# Autodesk Inventor assembly: arpans version robot
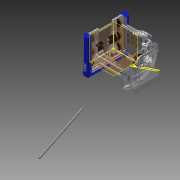
[picture p0: Inventor's stored thumbnail of the model, 180x180]
Saved by Autodesk Inventor 2013 (Build 170138000, 138)
## iProperties
Created: 2013-01-06
Part Number: arpans version robot
Document SubType Name: Assembly
Designer: Moses
Mass: 53939.9 g
Surface Area: 135947 cm^2
Volume: 43150 cm^3
Density: 1.25005 g/cm^3
Author: Moses
## Documents named in this file (39)
- C:\Users\Arpan\Documents\GitHub\frc2013CAD\arpans version robot.iam
- C:\Users\Arpan\Documents\GitHub\frc2013CAD\Drivetrain\Bearings\fr8zz-hex.ipt
- C:\Users\Arpan\Documents\GitHub\frc2013CAD\Drivetrain\Drive Wheel Assembly V2.iam
- C:\Users\Arpan\Documents\GitHub\frc2013CAD\Drivetrain\Standard Wheel Assembly V2.iam
- C:\Users\Arpan\Documents\GitHub\frc2013CAD\Drivetrain\Toughbox-mini\Toughbox-mini-hex-long.iam
- C:\Users\Arpan\Documents\GitHub\frc2013CAD\Drivetrain\6157K140 Shaft Collar\6157K140.ipt
- C:\Users\Arpan\Documents\GitHub\frc2013CAD\Drivetrain\Shaft Spacer Part1.ipt
- C:\Users\Arpan\Documents\GitHub\frc2013CAD\Drivetrain\Shaft Spacer Part2.ipt
- C:\Users\Arpan\Documents\GitHub\frc2013CAD\Drivetrain\Shaft Spacer Part3.ipt
- C:\Users\Arpan\Documents\GitHub\frc2013CAD\Drivetrain\Shaft Spacer Part4.ipt
- C:\Users\Arpan\Documents\GitHub\frc2013CAD\Drivetrain\Shaft Spacer Part5.ipt
- C:\Users\Arpan\Documents\GitHub\frc2013CAD\Drivetrain\Shaft Spacer Part6.ipt
- C:\Users\Arpan\Documents\GitHub\frc2013CAD\Drivetrain\6061K130 Shaft\6061K130.ipt
- C:\Users\Arpan\Documents\GitHub\frc2013CAD\Electrical\CS_compactRIO_cRIO-FRC-II.ipt
- C:\Users\Arpan\Documents\GitHub\frc2013CAD\Electrical\CS_WirelessBridge_DAP1522.ipt
- C:\Users\Arpan\Documents\GitHub\frc2013CAD\Drivetrain\Pneumatic_Compressor_VIAIR_00090\Pneumatic_Compressor_VIAIR_00090.iam
- C:\Users\Arpan\Documents\GitHub\frc2013CAD\Drivetrain\Mounting Bracket V1.500 - (toughbox-mini - sheet metal).ipt
- C:\Users\Arpan\Documents\GitHub\frc2013CAD\Drivetrain\Mounting Bracket V1.500 - (toughbox-mini - sheet metal - underside).ipt
- C:\Users\Arpan\Documents\GitHub\frc2013CAD\Drivetrain\Bearing Block V1.500 Drivetrain.ipt
- C:\Users\Arpan\Documents\GitHub\frc2013CAD\Drivetrain\Shaft Mount V1.500 Drivetrain.ipt
- C:\Users\Arpan\Documents\GitHub\frc2013CAD\Launcher\Shooter\Shooter Assembly v2.iam
- C:\Users\Arpan\Documents\GitHub\frc2013CAD\Chassis\Chassis Assembly 26x28 Version\Chassis Assembly 26x28 Version.iam
- C:\Users\Arpan\Documents\GitHub\frc2013CAD\Chassis\Bumpers\Bumper Assembly1 (26x28 robot).iam
- C:\Users\Arpan\Documents\GitHub\frc2013CAD\Electrical\Mounting Board 3.ipt
- C:\Users\Arpan\Documents\GitHub\frc2013CAD\Drivetrain\Wheel Mount Support Plate - drive wheel.ipt
- C:\Users\Arpan\Documents\GitHub\frc2013CAD\Drivetrain\Wheel Mount Support Plate.ipt
- C:\Users\Arpan\Documents\GitHub\frc2013CAD\Chassis\Bumpers\Bumper Assembly2 (26x28 robot).iam
- C:\Users\Arpan\Documents\GitHub\frc2013CAD\Chassis\Bumpers\Bumper Assembly3 (26x28 robot).iam
- C:\Users\Arpan\Documents\GitHub\frc2013CAD\Chassis\Bumpers\Bumper Assembly4 (26x28 robot).iam
- C:\Users\Arpan\Documents\GitHub\frc2013CAD\Electrical\Electrical Board 1.iam
- C:\Users\Arpan\Documents\GitHub\frc2013CAD\Cimber actual\Part4.ipt
- C:\Users\Arpan\Documents\GitHub\frc2013CAD\Cimber actual\tube v.iam
- C:\Users\Arpan\Documents\GitHub\frc2013CAD\Cimber actual\winch mount back support.ipt
- C:\Users\Arpan\Documents\GitHub\frc2013CAD\Cimber actual\ninja.ipt
- C:\Users\Arpan\Documents\GitHub\frc2013CAD\Electrical\ELEC_Battery_NP18-12B.iam
- C:\Users\Arpan\Documents\GitHub\frc2013CAD\M-Climber\M - Climber.iam
- C:\Users\Arpan\Documents\GitHub\frc2013CAD\Midwest Climber\Right Hook Whole Assembly_v2.iam
- C:\Users\Arpan\Documents\GitHub\frc2013CAD\Midwest Climber\Left Hook Whole Assembly_v2.iam
- C:\Users\Arpan\Documents\GitHub\frc2013CAD\Midwest Climber\Pyramid Pole.ipt
## Components (76 placed, 38 different names)
1. Chassis Assembly 26x28 Version:1 [sub-assembly] — Mate:1, Flush:1, Mate:2, Flush:4, Mate:3, Mate:4, Mate:5, Mate:8, Mate:9, Mate:10, Mate:17, Mate:18, Mate:19, Mate:20, Mate:21, Mate:26, Mate:27, Mate:28, Mate:29, Mate:34, Mate:35, Mate:36, Mate:37, Mate:42, Mate:43, Mate:44, Mate:47, Mate:48, Mate:51, Mate:52, Mate:55, Mate:83, Mate:84, Mate:85, Mate:89, Mate:98, Mate:99, Mate:100, Mate:101, Mate:115, Mate:116, Mate:117, Mate:118, Mate:119, Mate:120, Mate:125, Mate:126, Mate:127, Mate:128, Mate:129, Mate:130, Mate:132, Mate:136, Mate:153, Flush:17, Mate:154, Mate:159, Mate:190, Flush:162, Flush:191, Mate:194, Mate:195, Mate:196, Mate:197, Mate:198, Mate:199, Mate:200, Mate:201, Mate:202, Mate:203, Mate:204, Mate:205, Mate:206, Mate:207, Mate:208, Mate:209, Mate:210, Mate:211, Mate:212, Mate:213, Mate:214, Mate:215, Mate:216, Mate:217, Mate:218, Mate:219, Mate:220, Mate:221, Mate:222, Mate:223, Angle:4, Angle:5, Flush:222, Mate:312, Flush:233, Mate:316, Mate:317, Flush:235, Mate:331, Mate:332, Mate:333, Angle:13, Mate:340
2. Part4:1
3. tube v:1 [sub-assembly] — Flush:222
4. winch mount back support:1 — Mate:312, Flush:233
5. ninja:1 — Mate:317, Flush:235
6. winch mount back support:2 — Mate:316
7. M - Climber:1 [sub-assembly] — Angle:13, Mate:340
8. Right Hook Whole Assembly_v2:1 [sub-assembly] — Mate:351, Angle:15, Flush:246, Flush:248, Tangent:5, Tangent:8, Mate:354, Flush:250
9. Left Hook Whole Assembly_v2:1 [sub-assembly] — Flush:246, Tangent:4, Tangent:7, Mate:355, Flush:249, Flush:250
10. Pyramid Pole:1 — Tangent:4, Tangent:5, Tangent:7, Tangent:8
11. Bumper Assembly1 (26x28 robot):1 [sub-assembly] — Mate:5, Mate:3, Flush:6, Flush:9, Flush:10
12. Bumper Assembly1 (26x28 robot):2 [sub-assembly] — Mate:1, Flush:1, Flush:3, Flush:2, Flush:7, Flush:8
13. Bumper Assembly2 (26x28 robot):1 [sub-assembly] — Mate:2, Flush:2, Flush:3, Flush:4, Mate:5, Flush:10
14. Bumper Assembly3 (26x28 robot):1 [sub-assembly] — Flush:9, Mate:5, Flush:6
15. Bumper Assembly4 (26x28 robot):1 [sub-assembly] — Mate:4, Flush:7, Flush:8
16. Wheel Mount Support Plate - drive wheel:1 — Mate:194, Mate:195, Mate:196
17. Wheel Mount Support Plate - drive wheel:2 — Mate:197, Mate:198, Mate:199
18. Wheel Mount Support Plate:1 — Mate:200, Mate:201, Mate:202
19. Wheel Mount Support Plate:2 — Mate:203, Mate:204, Mate:205
20. Wheel Mount Support Plate:3 — Mate:206, Mate:207, Mate:208
21. Wheel Mount Support Plate:4 — Mate:209, Mate:210, Mate:211
22. Wheel Mount Support Plate:5 — Mate:212, Mate:213, Mate:214
23. Wheel Mount Support Plate:6 — Mate:215, Mate:216, Mate:217
24. Wheel Mount Support Plate:7 — Mate:218, Mate:219, Mate:220
25. Wheel Mount Support Plate:8 — Mate:221, Mate:222, Mate:223
26. Pneumatic_Compressor_VIAIR_00090:1 [sub-assembly] — Mate:144, Mate:240, Mate:241, Mate:244, Mate:245
27. Shaft Spacer Part1:1 — Insert:111
28. Shaft Spacer Part2:1 — Insert:112
29. Shaft Spacer Part1:3 — Insert:113
30. Shaft Spacer Part2:2 — Insert:114
31. Shaft Spacer Part3:1 — Insert:115
32. Shaft Spacer Part3:2 — Insert:116
33. Shaft Spacer Part4:2 — Insert:117
34. Shaft Spacer Part4:1 — Insert:118
35. Shaft Spacer Part5:1 — Insert:119
36. Shaft Spacer Part5:2 — Insert:120
37. Shaft Spacer Part6:1 — Insert:121
38. Shaft Spacer Part6:2 — Insert:122
39. 6157K140:1 — Insert:107, Insert:113
40. 6157K140:2 — Insert:108, Insert:114
41. 6157K140:3 — Insert:110, Insert:111
42. 6157K140:4 — Insert:109, Insert:112
43. Toughbox-mini-hex-long:2 [sub-assembly] — Mate:131, Mate:132, Mate:133, Mate:134, Mate:135, Insert:118
44. Toughbox-mini-hex-long:1 [sub-assembly] — Mate:136, Mate:137, Mate:138, Mate:139, Mate:140, Insert:117
45. fr8zz-hex:1 — Insert:94, Insert:116
46. Bearing Block V1.500 Drivetrain:1 — Mate:83, Mate:84, Mate:85, Insert:106
47. Bearing Block V1.500 Drivetrain:2 — Mate:98, Mate:99, Mate:100, Insert:94
48. fr8zz-hex:2 — Insert:106, Insert:115
49. Mounting Bracket V1.500 - (toughbox-mini - sheet metal):1 — Mate:115, Mate:116, Mate:117, Mate:137, Mate:138
50. Mounting Bracket V1.500 - (toughbox-mini - sheet metal):2 — Mate:118, Mate:119, Mate:120, Mate:131, Mate:133
51. Mounting Bracket V1.500 - (toughbox-mini - sheet metal - underside):1 — Mate:125, Mate:126, Mate:127
52. Mounting Bracket V1.500 - (toughbox-mini - sheet metal - underside):2 — Mate:128, Mate:129, Mate:130
53. Shaft Mount V1.500 Drivetrain:8 — Mate:34, Mate:35, Mate:51, Insert:121
54. Shaft Mount V1.500 Drivetrain:7 — Mate:28, Mate:29, Mate:48, Insert:110
55. Shaft Mount V1.500 Drivetrain:6 — Mate:42, Mate:43, Mate:47, Insert:122
56. Shaft Mount V1.500 Drivetrain:5 — Mate:36, Mate:37, Mate:44, Insert:107
57. Shaft Mount V1.500 Drivetrain:4 — Mate:26, Mate:27, Mate:55, Insert:7, Insert:109
58. Shaft Mount V1.500 Drivetrain:3 — Mate:20, Mate:21, Mate:52, Insert:5, Insert:119
59. Shaft Mount V1.500 Drivetrain:2 — Mate:17, Mate:18, Mate:19, Insert:2, Insert:108
60. Shaft Mount V1.500 Drivetrain:1 — Mate:8, Mate:9, Mate:10, Insert:1, Insert:120
61. 6061K130:4 — Insert:7, Mate:21
62. 6061K130:3 — Insert:5, Mate:22
63. 6061K130:2 — Insert:2, Mate:19
64. 6061K130:1 — Insert:1, Mate:17
65. Standard Wheel Assembly V2:3 [sub-assembly] — Mate:17, Flush:13, Rotation:1
66. Drive Wheel Assembly V2:1 [sub-assembly] — Mate:89, Flush:13, Flush:15, Mate:139, Mate:140, Rotation:1, Rotation:2, Tangent:3
67. Standard Wheel Assembly V2:1 [sub-assembly] — Mate:19, Flush:15, Rotation:2
68. Standard Wheel Assembly V2:2 [sub-assembly] — Mate:21, Flush:11, Rotation:4
69. Standard Wheel Assembly V2:4 [sub-assembly] — Mate:22, Flush:12, Rotation:3
70. Drive Wheel Assembly V2:2 [sub-assembly] — Mate:101, Flush:11, Flush:12, Mate:134, Mate:135, Rotation:3, Rotation:4
71. ELEC_Battery_NP18-12B:1 [sub-assembly] — Mate:331, Mate:332, Mate:333
72. Mounting Board 3:1 — Mate:190, Flush:162, Mate:16, Mate:188, Mate:189, Flush:191, Mate:144, Mate:240, Mate:241, Mate:244, Mate:245
73. Electrical Board 1:1 [sub-assembly] — Mate:242, Mate:243, Flush:192
74. CS_WirelessBridge_DAP1522:1 — Flush:152, Mate:164, Flush:224
75. CS_compactRIO_cRIO-FRC-II:1 — Mate:16, Mate:188, Mate:189
76. Shooter Assembly v2:1 [sub-assembly] — Mate:153, Flush:17, Mate:154, Mate:159, Mate:164, Flush:152, Flush:224, Mate:242, Mate:243, Flush:192, Mate:351, Angle:15, Flush:248, Mate:354, Mate:355, Flush:249
## Relationships (180: Mate 119, Flush 26, Insert 22, Tangent 5, RelateRotation 4, Angle 4)
- Mate:1: Chassis Assembly 26x28 Version:1 ↔ Bumper Assembly1 (26x28 robot):2
- Flush:1: Chassis Assembly 26x28 Version:1 ↔ Bumper Assembly1 (26x28 robot):2
- Mate:2: Chassis Assembly 26x28 Version:1 ↔ Bumper Assembly2 (26x28 robot):1
- Flush:2: Bumper Assembly1 (26x28 robot):2 ↔ Bumper Assembly2 (26x28 robot):1
- Flush:3: Bumper Assembly1 (26x28 robot):2 ↔ Bumper Assembly2 (26x28 robot):1
- Flush:4 (-69.85 mm): Chassis Assembly 26x28 Version:1 ↔ Bumper Assembly2 (26x28 robot):1
- Mate:5: Bumper Assembly1 (26x28 robot):1 ↔ Bumper Assembly2 (26x28 robot):1
- Mate:3: Chassis Assembly 26x28 Version:1 ↔ Bumper Assembly1 (26x28 robot):1
- Flush:6: Bumper Assembly1 (26x28 robot):1 ↔ Bumper Assembly3 (26x28 robot):1
- Mate:4: Chassis Assembly 26x28 Version:1 ↔ Bumper Assembly4 (26x28 robot):1
- Flush:7: Bumper Assembly1 (26x28 robot):2 ↔ Bumper Assembly4 (26x28 robot):1
- Flush:8: Bumper Assembly1 (26x28 robot):2 ↔ Bumper Assembly4 (26x28 robot):1
- Flush:9: Bumper Assembly1 (26x28 robot):1 ↔ Bumper Assembly3 (26x28 robot):1
- Flush:10: Bumper Assembly1 (26x28 robot):1 ↔ Bumper Assembly2 (26x28 robot):1
- Mate:5: Chassis Assembly 26x28 Version:1 ↔ Bumper Assembly3 (26x28 robot):1
- Insert:1 (-6.35 mm): Shaft Mount V1.500 Drivetrain:1 ↔ 6061K130:1
- Insert:2 (-6.35 mm): Shaft Mount V1.500 Drivetrain:2 ↔ 6061K130:2
- Insert:5 (-6.35 mm): Shaft Mount V1.500 Drivetrain:3 ↔ 6061K130:3
- Insert:7 (-6.35 mm): Shaft Mount V1.500 Drivetrain:4 ↔ 6061K130:4
- Mate:8: Chassis Assembly 26x28 Version:1 ↔ Shaft Mount V1.500 Drivetrain:1
- Mate:9: Chassis Assembly 26x28 Version:1 ↔ Shaft Mount V1.500 Drivetrain:1
- Mate:10: Chassis Assembly 26x28 Version:1 ↔ Shaft Mount V1.500 Drivetrain:1
- Mate:17: Chassis Assembly 26x28 Version:1 ↔ Shaft Mount V1.500 Drivetrain:2
- Mate:18: Chassis Assembly 26x28 Version:1 ↔ Shaft Mount V1.500 Drivetrain:2
- Mate:19: Chassis Assembly 26x28 Version:1 ↔ Shaft Mount V1.500 Drivetrain:2
- Mate:20: Chassis Assembly 26x28 Version:1 ↔ Shaft Mount V1.500 Drivetrain:3
- Mate:21: Chassis Assembly 26x28 Version:1 ↔ Shaft Mount V1.500 Drivetrain:3
- Mate:26: Chassis Assembly 26x28 Version:1 ↔ Shaft Mount V1.500 Drivetrain:4
- Mate:27: Chassis Assembly 26x28 Version:1 ↔ Shaft Mount V1.500 Drivetrain:4
- Mate:28: Chassis Assembly 26x28 Version:1 ↔ Shaft Mount V1.500 Drivetrain:7
- Mate:29: Chassis Assembly 26x28 Version:1 ↔ Shaft Mount V1.500 Drivetrain:7
- Mate:34: Chassis Assembly 26x28 Version:1 ↔ Shaft Mount V1.500 Drivetrain:8
- Mate:35: Chassis Assembly 26x28 Version:1 ↔ Shaft Mount V1.500 Drivetrain:8
- Mate:36: Chassis Assembly 26x28 Version:1 ↔ Shaft Mount V1.500 Drivetrain:5
- Mate:37: Chassis Assembly 26x28 Version:1 ↔ Shaft Mount V1.500 Drivetrain:5
- Mate:42: Chassis Assembly 26x28 Version:1 ↔ Shaft Mount V1.500 Drivetrain:6
- Mate:43: Chassis Assembly 26x28 Version:1 ↔ Shaft Mount V1.500 Drivetrain:6
- Mate:44: Chassis Assembly 26x28 Version:1 ↔ Shaft Mount V1.500 Drivetrain:5
- Mate:47: Chassis Assembly 26x28 Version:1 ↔ Shaft Mount V1.500 Drivetrain:6
- Mate:48: Chassis Assembly 26x28 Version:1 ↔ Shaft Mount V1.500 Drivetrain:7
- Mate:51: Chassis Assembly 26x28 Version:1 ↔ Shaft Mount V1.500 Drivetrain:8
- Mate:52: Chassis Assembly 26x28 Version:1 ↔ Shaft Mount V1.500 Drivetrain:3
- Mate:55: Chassis Assembly 26x28 Version:1 ↔ Shaft Mount V1.500 Drivetrain:4
- Mate:17: 6061K130:1 ↔ Standard Wheel Assembly V2:3
- Mate:19: 6061K130:2 ↔ Standard Wheel Assembly V2:1
- Mate:21: 6061K130:4 ↔ Standard Wheel Assembly V2:2
- Mate:22: 6061K130:3 ↔ Standard Wheel Assembly V2:4
- Mate:83: Chassis Assembly 26x28 Version:1 ↔ Bearing Block V1.500 Drivetrain:1
- Mate:84: Chassis Assembly 26x28 Version:1 ↔ Bearing Block V1.500 Drivetrain:1
- Mate:85: Chassis Assembly 26x28 Version:1 ↔ Bearing Block V1.500 Drivetrain:1
- Mate:89 (6.35 mm): Chassis Assembly 26x28 Version:1 ↔ Drive Wheel Assembly V2:1
- Insert:94: fr8zz-hex:1 ↔ Bearing Block V1.500 Drivetrain:2
- Mate:98: Chassis Assembly 26x28 Version:1 ↔ Bearing Block V1.500 Drivetrain:2
- Mate:99: Chassis Assembly 26x28 Version:1 ↔ Bearing Block V1.500 Drivetrain:2
- Mate:100: Chassis Assembly 26x28 Version:1 ↔ Bearing Block V1.500 Drivetrain:2
- Mate:101 (6.35 mm): Chassis Assembly 26x28 Version:1 ↔ Drive Wheel Assembly V2:2
- Insert:106: Bearing Block V1.500 Drivetrain:1 ↔ fr8zz-hex:2
- Mate:115: Chassis Assembly 26x28 Version:1 ↔ Mounting Bracket V1.500 - (toughbox-mini - sheet metal):1
- Mate:116: Chassis Assembly 26x28 Version:1 ↔ Mounting Bracket V1.500 - (toughbox-mini - sheet metal):1
- Mate:117: Chassis Assembly 26x28 Version:1 ↔ Mounting Bracket V1.500 - (toughbox-mini - sheet metal):1
- Mate:118: Chassis Assembly 26x28 Version:1 ↔ Mounting Bracket V1.500 - (toughbox-mini - sheet metal):2
- Mate:119: Chassis Assembly 26x28 Version:1 ↔ Mounting Bracket V1.500 - (toughbox-mini - sheet metal):2
- Mate:120: Chassis Assembly 26x28 Version:1 ↔ Mounting Bracket V1.500 - (toughbox-mini - sheet metal):2
- Flush:11: Standard Wheel Assembly V2:2 ↔ Drive Wheel Assembly V2:2
- Flush:12: Standard Wheel Assembly V2:4 ↔ Drive Wheel Assembly V2:2
- Flush:13: Standard Wheel Assembly V2:3 ↔ Drive Wheel Assembly V2:1
- Mate:125: Chassis Assembly 26x28 Version:1 ↔ Mounting Bracket V1.500 - (toughbox-mini - sheet metal - underside):1
- Mate:126: Chassis Assembly 26x28 Version:1 ↔ Mounting Bracket V1.500 - (toughbox-mini - sheet metal - underside):1
- Mate:127: Chassis Assembly 26x28 Version:1 ↔ Mounting Bracket V1.500 - (toughbox-mini - sheet metal - underside):1
- Mate:128: Chassis Assembly 26x28 Version:1 ↔ Mounting Bracket V1.500 - (toughbox-mini - sheet metal - underside):2
- Mate:129: Chassis Assembly 26x28 Version:1 ↔ Mounting Bracket V1.500 - (toughbox-mini - sheet metal - underside):2
- Mate:130: Chassis Assembly 26x28 Version:1 ↔ Mounting Bracket V1.500 - (toughbox-mini - sheet metal - underside):2
- Flush:15: Drive Wheel Assembly V2:1 ↔ Standard Wheel Assembly V2:1
- Mate:131: Toughbox-mini-hex-long:2 ↔ Mounting Bracket V1.500 - (toughbox-mini - sheet metal):2
- Mate:132: Chassis Assembly 26x28 Version:1 ↔ Toughbox-mini-hex-long:2
- Mate:133: Toughbox-mini-hex-long:2 ↔ Mounting Bracket V1.500 - (toughbox-mini - sheet metal):2
- Mate:134: Toughbox-mini-hex-long:2 ↔ Drive Wheel Assembly V2:2
- Mate:135: Toughbox-mini-hex-long:2 ↔ Drive Wheel Assembly V2:2
- Mate:136: Chassis Assembly 26x28 Version:1 ↔ Toughbox-mini-hex-long:1
- Mate:137: Toughbox-mini-hex-long:1 ↔ Mounting Bracket V1.500 - (toughbox-mini - sheet metal):1
- Mate:138: Toughbox-mini-hex-long:1 ↔ Mounting Bracket V1.500 - (toughbox-mini - sheet metal):1
- Mate:139: Toughbox-mini-hex-long:1 ↔ Drive Wheel Assembly V2:1
- Mate:140: Toughbox-mini-hex-long:1 ↔ Drive Wheel Assembly V2:1
- Rotation:1 [RelateRotation] (1 ul): Standard Wheel Assembly V2:3 ↔ Drive Wheel Assembly V2:1
- Rotation:2 [RelateRotation] (1 ul): Drive Wheel Assembly V2:1 ↔ Standard Wheel Assembly V2:1
- Rotation:3 [RelateRotation] (1 ul): Standard Wheel Assembly V2:4 ↔ Drive Wheel Assembly V2:2
- Rotation:4 [RelateRotation] (1 ul): Standard Wheel Assembly V2:2 ↔ Drive Wheel Assembly V2:2
- Insert:107: 6157K140:1 ↔ Shaft Mount V1.500 Drivetrain:5
- Insert:108: 6157K140:2 ↔ Shaft Mount V1.500 Drivetrain:2
- Insert:109: 6157K140:4 ↔ Shaft Mount V1.500 Drivetrain:4
- Insert:110: 6157K140:3 ↔ Shaft Mount V1.500 Drivetrain:7
- Insert:111: Shaft Spacer Part1:1 ↔ 6157K140:3
- Insert:112: Shaft Spacer Part2:1 ↔ 6157K140:4
- Insert:113: Shaft Spacer Part1:3 ↔ 6157K140:1
- Insert:114: Shaft Spacer Part2:2 ↔ 6157K140:2
- Insert:115: Shaft Spacer Part3:1 ↔ fr8zz-hex:2
- Insert:116: Shaft Spacer Part3:2 ↔ fr8zz-hex:1
- Insert:117: Shaft Spacer Part4:2 ↔ Toughbox-mini-hex-long:1
- Insert:118: Shaft Spacer Part4:1 ↔ Toughbox-mini-hex-long:2
- Insert:119: Shaft Spacer Part5:1 ↔ Shaft Mount V1.500 Drivetrain:3
- Insert:120: Shaft Spacer Part5:2 ↔ Shaft Mount V1.500 Drivetrain:1
- Insert:121: Shaft Spacer Part6:1 ↔ Shaft Mount V1.500 Drivetrain:8
- Insert:122: Shaft Spacer Part6:2 ↔ Shaft Mount V1.500 Drivetrain:6
- Mate:16: Mounting Board 3:1 ↔ CS_compactRIO_cRIO-FRC-II:1
- Mate:144: Pneumatic_Compressor_VIAIR_00090:1 ↔ Mounting Board 3:1
- Flush:152: CS_WirelessBridge_DAP1522:1 ↔ Shooter Assembly v2:1
- Mate:153: Chassis Assembly 26x28 Version:1 ↔ Shooter Assembly v2:1
- Flush:17: Chassis Assembly 26x28 Version:1 ↔ Shooter Assembly v2:1
- Mate:154: Chassis Assembly 26x28 Version:1 ↔ Shooter Assembly v2:1
- Mate:159: Chassis Assembly 26x28 Version:1 ↔ Shooter Assembly v2:1
- Mate:164: CS_WirelessBridge_DAP1522:1 ↔ Shooter Assembly v2:1
- Mate:188: Mounting Board 3:1 ↔ CS_compactRIO_cRIO-FRC-II:1
- Mate:189: Mounting Board 3:1 ↔ CS_compactRIO_cRIO-FRC-II:1
- Mate:190: Chassis Assembly 26x28 Version:1 ↔ Mounting Board 3:1
- Flush:162: Chassis Assembly 26x28 Version:1 ↔ Mounting Board 3:1
- Flush:191: Chassis Assembly 26x28 Version:1 ↔ Mounting Board 3:1
- Mate:194: Chassis Assembly 26x28 Version:1 ↔ Wheel Mount Support Plate - drive wheel:1
- Mate:195: Chassis Assembly 26x28 Version:1 ↔ Wheel Mount Support Plate - drive wheel:1
- Mate:196: Chassis Assembly 26x28 Version:1 ↔ Wheel Mount Support Plate - drive wheel:1
- Mate:197: Chassis Assembly 26x28 Version:1 ↔ Wheel Mount Support Plate - drive wheel:2
- Mate:198: Chassis Assembly 26x28 Version:1 ↔ Wheel Mount Support Plate - drive wheel:2
- Mate:199: Chassis Assembly 26x28 Version:1 ↔ Wheel Mount Support Plate - drive wheel:2
- Mate:200: Chassis Assembly 26x28 Version:1 ↔ Wheel Mount Support Plate:1
- Mate:201: Chassis Assembly 26x28 Version:1 ↔ Wheel Mount Support Plate:1
- Mate:202: Chassis Assembly 26x28 Version:1 ↔ Wheel Mount Support Plate:1
- Mate:203: Chassis Assembly 26x28 Version:1 ↔ Wheel Mount Support Plate:2
- Mate:204: Chassis Assembly 26x28 Version:1 ↔ Wheel Mount Support Plate:2
- Mate:205: Chassis Assembly 26x28 Version:1 ↔ Wheel Mount Support Plate:2
- Mate:206: Chassis Assembly 26x28 Version:1 ↔ Wheel Mount Support Plate:3
- Mate:207: Chassis Assembly 26x28 Version:1 ↔ Wheel Mount Support Plate:3
- Mate:208: Chassis Assembly 26x28 Version:1 ↔ Wheel Mount Support Plate:3
- Mate:209: Chassis Assembly 26x28 Version:1 ↔ Wheel Mount Support Plate:4
- Mate:210: Chassis Assembly 26x28 Version:1 ↔ Wheel Mount Support Plate:4
- Mate:211: Chassis Assembly 26x28 Version:1 ↔ Wheel Mount Support Plate:4
- Mate:212: Chassis Assembly 26x28 Version:1 ↔ Wheel Mount Support Plate:5
- Mate:213: Chassis Assembly 26x28 Version:1 ↔ Wheel Mount Support Plate:5
- Mate:214: Chassis Assembly 26x28 Version:1 ↔ Wheel Mount Support Plate:5
- Mate:215: Chassis Assembly 26x28 Version:1 ↔ Wheel Mount Support Plate:6
- Mate:216: Chassis Assembly 26x28 Version:1 ↔ Wheel Mount Support Plate:6
- Mate:217: Chassis Assembly 26x28 Version:1 ↔ Wheel Mount Support Plate:6
- Mate:218: Chassis Assembly 26x28 Version:1 ↔ Wheel Mount Support Plate:7
- Mate:219: Chassis Assembly 26x28 Version:1 ↔ Wheel Mount Support Plate:7
- Mate:220: Chassis Assembly 26x28 Version:1 ↔ Wheel Mount Support Plate:7
- Mate:221: Chassis Assembly 26x28 Version:1 ↔ Wheel Mount Support Plate:8
- Mate:222: Chassis Assembly 26x28 Version:1 ↔ Wheel Mount Support Plate:8
- Mate:223: Chassis Assembly 26x28 Version:1 ↔ Wheel Mount Support Plate:8
- Flush:224: CS_WirelessBridge_DAP1522:1 ↔ Shooter Assembly v2:1
- Mate:240: Pneumatic_Compressor_VIAIR_00090:1 ↔ Mounting Board 3:1
- Mate:241: Pneumatic_Compressor_VIAIR_00090:1 ↔ Mounting Board 3:1
- Mate:242 (12.7 mm): Electrical Board 1:1 ↔ Shooter Assembly v2:1
- Mate:243: Electrical Board 1:1 ↔ Shooter Assembly v2:1
- Flush:192: Electrical Board 1:1 ↔ Shooter Assembly v2:1
- Mate:244: Pneumatic_Compressor_VIAIR_00090:1 ↔ Mounting Board 3:1
- Mate:245: Pneumatic_Compressor_VIAIR_00090:1 ↔ Mounting Board 3:1
- Angle:4 (0 deg): Chassis Assembly 26x28 Version:1
- Angle:5 (0 deg): Chassis Assembly 26x28 Version:1
- Tangent:3: Drive Wheel Assembly V2:1
- Flush:222: Chassis Assembly 26x28 Version:1 ↔ tube v:1
- Mate:312: Chassis Assembly 26x28 Version:1 ↔ winch mount back support:1
- Flush:233: Chassis Assembly 26x28 Version:1 ↔ winch mount back support:1
- Mate:316: Chassis Assembly 26x28 Version:1 ↔ winch mount back support:2
- Mate:317: Chassis Assembly 26x28 Version:1 ↔ ninja:1
- Flush:235: Chassis Assembly 26x28 Version:1 ↔ ninja:1
- Mate:331: Chassis Assembly 26x28 Version:1 ↔ ELEC_Battery_NP18-12B:1
- Mate:332: Chassis Assembly 26x28 Version:1 ↔ ELEC_Battery_NP18-12B:1
- Mate:333: Chassis Assembly 26x28 Version:1 ↔ ELEC_Battery_NP18-12B:1
- Angle:13 (120 deg): Chassis Assembly 26x28 Version:1 ↔ M - Climber:1
- Mate:340 (47.625 mm): Chassis Assembly 26x28 Version:1 ↔ M - Climber:1
- Mate:351 (19.05 mm): Right Hook Whole Assembly_v2:1 ↔ Shooter Assembly v2:1
- Angle:15 (0 deg): Right Hook Whole Assembly_v2:1 ↔ Shooter Assembly v2:1
- Flush:246: Right Hook Whole Assembly_v2:1 ↔ Left Hook Whole Assembly_v2:1
- Flush:248: Right Hook Whole Assembly_v2:1 ↔ Shooter Assembly v2:1
- Tangent:4: Left Hook Whole Assembly_v2:1 ↔ Pyramid Pole:1
- Tangent:5: Right Hook Whole Assembly_v2:1 ↔ Pyramid Pole:1
- Tangent:7: Left Hook Whole Assembly_v2:1 ↔ Pyramid Pole:1
- Tangent:8: Right Hook Whole Assembly_v2:1 ↔ Pyramid Pole:1
- Mate:354: Right Hook Whole Assembly_v2:1 ↔ Shooter Assembly v2:1
- Mate:355 (19.05 mm): Left Hook Whole Assembly_v2:1 ↔ Shooter Assembly v2:1
- Flush:249: Left Hook Whole Assembly_v2:1 ↔ Shooter Assembly v2:1
- Flush:250: Right Hook Whole Assembly_v2:1 ↔ Left Hook Whole Assembly_v2:1
